# Autodesk Inventor assembly: 3606-0000-0096 assembly
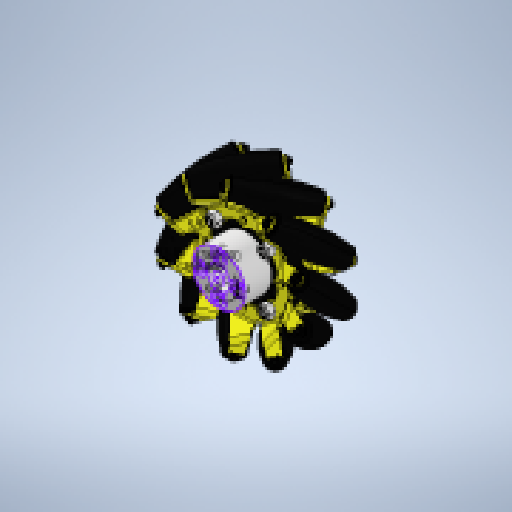
[picture p0: Inventor's stored thumbnail of the model, 512x512]
Saved by Autodesk Inventor 2023 (Build 270158000, 158)
## iProperties
Created: 2020-12-01
Part Number: 3606-0000-0096 assembly
Description: STEP AP203
Document SubType Name: Assembly
Designer: TakeHomePC
Sending System: SolidWorks 2016
Preprocessor: SwSTEP 2.0
Title: 3606-0000-0096 assembly not joined.STEP
Revision Number: ANY
## iProperties of the stored document MemberDocs/xGmfnv1wmH0wodwrzN1areal1La
Created: 2020-12-01
Part Number: 3606-0000-0096 assembly
Description: STEP AP203
Document SubType Name: Assembly
Designer: TakeHomePC
Sending System: SolidWorks 2016
Preprocessor: SwSTEP 2.0
Title: 3606-0000-0096 assembly not joined.STEP
Revision Number: ANY
## Documents named in this file (9)
- C:\Users\matt\Documents\Inventor\FTC\2022-23 FTC\Mech Chassis\GoBilda Mec Wheel\3213-3606-0002\3606-0000-0096 assembly.iam
- C:\Users\matt\Documents\Inventor\FTC\2022-23 FTC\Mech Chassis\GoBilda Mec Wheel\3213-3606-0002\3606-0000-0096 left slant side plate.ipt
- C:\Users\matt\Documents\Inventor\FTC\2022-23 FTC\Mech Chassis\GoBilda Mec Wheel\3213-3606-0002\3606-XXXX-0096 roller assembly.iam
- C:\Users\matt\Documents\Inventor\FTC\2022-23 FTC\Mech Chassis\GoBilda Mec Wheel\3213-3606-0002\2800-0004-0020_90128A207.ipt
- C:\Users\matt\Documents\Inventor\FTC\2022-23 FTC\Mech Chassis\GoBilda Mec Wheel\3213-3606-0002\2812-0004-0007_90576A103.ipt
- C:\Users\matt\Documents\Inventor\FTC\2022-23 FTC\Mech Chassis\GoBilda Mec Wheel\3213-3606-0002\3606-XXXX-0096 core.ipt
- C:\Users\matt\Documents\Inventor\FTC\2022-23 FTC\Mech Chassis\GoBilda Mech Hub 0500 Hex Spacer  inserts V2.ipt
- C:\Users\matt\Documents\Inventor\FTC\2022-23 FTC\Mech Chassis\GoBilda Mech Hub 0500 HexV2.ipt
- C:\Users\matt\Documents\Inventor\FTC\2022-23 FTC\Mech Chassis\3606-XXXX-0096 core.ipt
## Components (23 placed, 23 different names)
1. 3606-0000-0096 left slant side plate_1 — Mate:4, Mate:5, Mate:14, Mate:22
2. 3606-0000-0096 left slant side plate_2 — Mate:4, Mate:5, Mate:9, Mate:10, Mate:13, Mate:19, Mate:20, Mate:21, Mate:23
3. 3606-XXXX-0096 core_3 — Mate:19, Mate:20, Mate:21, Mate:22, Mate:24, Mate:27, Mate:28, Mate:29
4. 3606-XXXX-0096 roller assembly_4 [sub-assembly]
5. 3606-XXXX-0096 roller assembly_5 [sub-assembly]
6. 3606-XXXX-0096 roller assembly_6 [sub-assembly]
7. 3606-XXXX-0096 roller assembly_7 [sub-assembly]
8. 3606-XXXX-0096 roller assembly_8 [sub-assembly]
9. 3606-XXXX-0096 roller assembly_9 [sub-assembly]
10. 3606-XXXX-0096 roller assembly_10 [sub-assembly]
11. 3606-XXXX-0096 roller assembly_11 [sub-assembly]
12. 3606-XXXX-0096 roller assembly_12 [sub-assembly]
13. 3606-XXXX-0096 roller assembly_13 [sub-assembly]
14. 2800-0004-0020_90128A207_14 — Flush:1, Flush:2, Mate:13, Mate:16
15. 2812-0004-0007_90576A103_15 — Flush:4, Mate:18
16. 2812-0004-0007_90576A103_16 — Flush:6, Mate:14, Mate:15
17. 2812-0004-0007_90576A103_17 — Flush:5, Flush:6, Mate:16
18. 2812-0004-0007_90576A103_18 — Flush:4, Flush:5, Mate:17
19. 2800-0004-0020_90128A207_19 — Flush:2, Flush:3, Mate:17, Mate:24
20. 2800-0004-0020_90128A207_20 — Flush:3, Mate:9, Mate:10, Mate:15
21. 2800-0004-0020_90128A207_21 — Flush:1, Mate:18, Mate:23
22. GoBilda Mech Hub 0500 Hex Spacer  inserts V2:1 — Flush:7, Mate:29
23. GoBilda Mech Hub 0500 HexV2:1 — Mate:27, Mate:28, Flush:7
## Relationships (28: Mate 21, Flush 7)
- Mate:4: 3606-0000-0096 left slant side plate_1 ↔ 3606-0000-0096 left slant side plate_2
- Mate:5: 3606-0000-0096 left slant side plate_1 ↔ 3606-0000-0096 left slant side plate_2
- Flush:1: 2800-0004-0020_90128A207_14 ↔ 2800-0004-0020_90128A207_21
- Flush:2: 2800-0004-0020_90128A207_14 ↔ 2800-0004-0020_90128A207_19
- Flush:3: 2800-0004-0020_90128A207_19 ↔ 2800-0004-0020_90128A207_20
- Mate:9: 3606-0000-0096 left slant side plate_2 ↔ 2800-0004-0020_90128A207_20
- Mate:10: 3606-0000-0096 left slant side plate_2 ↔ 2800-0004-0020_90128A207_20
- Mate:13: 3606-0000-0096 left slant side plate_2 ↔ 2800-0004-0020_90128A207_14
- Flush:4: 2812-0004-0007_90576A103_15 ↔ 2812-0004-0007_90576A103_18
- Flush:5: 2812-0004-0007_90576A103_17 ↔ 2812-0004-0007_90576A103_18
- Flush:6: 2812-0004-0007_90576A103_16 ↔ 2812-0004-0007_90576A103_17
- Mate:14: 3606-0000-0096 left slant side plate_1 ↔ 2812-0004-0007_90576A103_16
- Mate:15: 2812-0004-0007_90576A103_16 ↔ 2800-0004-0020_90128A207_20
- Mate:16: 2800-0004-0020_90128A207_14 ↔ 2812-0004-0007_90576A103_17
- Mate:17: 2812-0004-0007_90576A103_18 ↔ 2800-0004-0020_90128A207_19
- Mate:18: 2812-0004-0007_90576A103_15 ↔ 2800-0004-0020_90128A207_21
- Mate:19: 3606-0000-0096 left slant side plate_2 ↔ 3606-XXXX-0096 core_3
- Mate:20: 3606-0000-0096 left slant side plate_2 ↔ 3606-XXXX-0096 core_3
- Mate:21: 3606-0000-0096 left slant side plate_2 ↔ 3606-XXXX-0096 core_3
- Mate:22: 3606-0000-0096 left slant side plate_1 ↔ 3606-XXXX-0096 core_3
- Mate:23: 3606-0000-0096 left slant side plate_2 ↔ 2800-0004-0020_90128A207_21
- Mate:24: 3606-XXXX-0096 core_3 ↔ 2800-0004-0020_90128A207_19
- [Mate]: 3606-XXXX-0096 core_3 ↔ GoBilda Mech Hub 0500 Hex Spacer  inserts V2:1
- [Mate]: 3606-XXXX-0096 core_3 ↔ GoBilda Mech Hub 0500 Hex Spacer  inserts V2:1
- Mate:27: 3606-XXXX-0096 core_3 ↔ GoBilda Mech Hub 0500 HexV2:1
- Mate:28: 3606-XXXX-0096 core_3 ↔ GoBilda Mech Hub 0500 HexV2:1
- Flush:7: GoBilda Mech Hub 0500 Hex Spacer  inserts V2:1 ↔ GoBilda Mech Hub 0500 HexV2:1
- Mate:29: 3606-XXXX-0096 core_3 ↔ GoBilda Mech Hub 0500 Hex Spacer  inserts V2:1
